# Autodesk Inventor assembly: EnsamblajeCarcaza
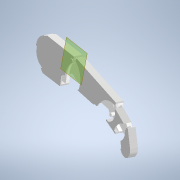
[picture p0: Inventor's stored thumbnail of the model, 180x180]
Saved by Autodesk Inventor 2022 (Build 260153000, 153)
## iProperties
Created: 2022-11-06
Part Number: EnsamblajeCarcaza
Document SubType Name: Assembly
Designer: Mauricio Guerrero
Author: Mauricio Guerrero
## Documents named in this file (9)
- C:\Users\Griselda Hernandez\Documents\FIME\7mo Semestre\Biomecanica\PIA\PiezasPIA\EnsamblajeCarcaza.iam
- C:\Users\Griselda Hernandez\Documents\FIME\7mo Semestre\Biomecanica\PIA\PiezasPIA\Pieza4.ipt
- C:\Users\Griselda Hernandez\Documents\FIME\7mo Semestre\Biomecanica\PIA\PiezasPIA\Pieza1.ipt
- C:\Users\Griselda Hernandez\Documents\FIME\7mo Semestre\Biomecanica\PIA\PiezasPIA\Pieza4_Carcasa.ipt
- C:\Users\Griselda Hernandez\Documents\FIME\7mo Semestre\Biomecanica\PIA\PiezasPIA\Pieza2.ipt
- C:\Users\Griselda Hernandez\Documents\FIME\7mo Semestre\Biomecanica\PIA\PiezasPIA\Pieza1_Carcasa.ipt
- C:\Users\Griselda Hernandez\Documents\FIME\7mo Semestre\Biomecanica\PIA\PiezasPIA\Pieza3.ipt
- C:\Users\Griselda Hernandez\Documents\FIME\7mo Semestre\Biomecanica\PIA\PiezasPIA\Pieza2_Carcasa.ipt
- C:\Users\Griselda Hernandez\Documents\FIME\7mo Semestre\Biomecanica\PIA\PiezasPIA\Pieza3_Carcasa.ipt
## Components (8 placed, 8 different names)
1. Pieza4:1 — Coincidencia:1, Coincidencia:2, Coincidencia:3, Coincidencia:5, Nivelación:1
2. Pieza1:1 — Coincidencia:1, Coincidencia:2, Coincidencia:6, Coincidencia:7, Coincidencia:8, Nivelación:2, Coincidencia:9
3. Pieza4_Carcasa:1 — Coincidencia:3, Coincidencia:5, Nivelación:1
4. Pieza2:1 — Coincidencia:6, Coincidencia:7, Coincidencia:10, Nivelación:3, Coincidencia:12, Coincidencia:13, Nivelación:4, Coincidencia:14, Coincidencia:15
5. Pieza1_Carcasa:1 — Coincidencia:8, Nivelación:2, Coincidencia:9
6. Pieza3:1 — Coincidencia:10, Coincidencia:15, Coincidencia:16, Nivelación:5, Coincidencia:17
7. Pieza2_Carcasa:1 — Nivelación:3, Coincidencia:12, Coincidencia:13, Nivelación:4, Coincidencia:14
8. Pieza3_Carcasa:1 — Coincidencia:16, Nivelación:5, Coincidencia:17
## Relationships (20: Mate 15, Flush 5)
- Coincidencia:1 [Mate]: Pieza4:1 ↔ Pieza1:1
- Coincidencia:2 [Mate]: Pieza4:1 ↔ Pieza1:1
- Coincidencia:3 [Mate]: Pieza4:1 ↔ Pieza4_Carcasa:1
- Coincidencia:5 [Mate]: Pieza4:1 ↔ Pieza4_Carcasa:1
- Nivelación:1 [Flush]: Pieza4:1 ↔ Pieza4_Carcasa:1
- Coincidencia:6 [Mate]: Pieza1:1 ↔ Pieza2:1
- Coincidencia:7 [Mate]: Pieza1:1 ↔ Pieza2:1
- Coincidencia:8 [Mate]: Pieza1:1 ↔ Pieza1_Carcasa:1
- Nivelación:2 [Flush]: Pieza1:1 ↔ Pieza1_Carcasa:1
- Coincidencia:9 [Mate]: Pieza1:1 ↔ Pieza1_Carcasa:1
- Coincidencia:10 [Mate]: Pieza2:1 ↔ Pieza3:1
- Nivelación:3 [Flush]: Pieza2:1 ↔ Pieza2_Carcasa:1
- Coincidencia:12 [Mate]: Pieza2:1 ↔ Pieza2_Carcasa:1
- Coincidencia:13 [Mate]: Pieza2:1 ↔ Pieza2_Carcasa:1
- Nivelación:4 [Flush]: Pieza2:1 ↔ Pieza2_Carcasa:1
- Coincidencia:14 [Mate]: Pieza2:1 ↔ Pieza2_Carcasa:1
- Coincidencia:15 [Mate]: Pieza2:1 ↔ Pieza3:1
- Coincidencia:16 [Mate]: Pieza3:1 ↔ Pieza3_Carcasa:1
- Nivelación:5 [Flush]: Pieza3:1 ↔ Pieza3_Carcasa:1
- Coincidencia:17 [Mate]: Pieza3:1 ↔ Pieza3_Carcasa:1
